# Autodesk Inventor assembly: P1704_E001
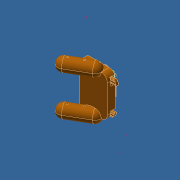
[picture p0: Inventor's stored thumbnail of the model, 180x180]
Saved by Autodesk Inventor 2019 (Build 230136000, 136)
## iProperties
Created: 2019-04-29
Part Number: P1704_E001
Material: Générique
Document SubType Name: Assembly
Designer: Joan.MAILLARD
Author: Joan.MAILLARD
## Documents named in this file (16)
- P:\projet_manette\manette\06_Dessins\2019\Manette universelle\P1704_E001.iam
- P:\projet_manette\manette\06_Dessins\2019\Manette universelle\P1704_004_mainDroiteExterieur.ipt
- P:\projet_manette\manette\06_Dessins\2019\Manette universelle\P1704_005_mainGaucheExterieur.ipt
- P:\projet_manette\manette\06_Dessins\2019\Manette universelle\P1704_001_basManette.ipt
- P:\projet_manette\manette\06_Dessins\2019\Manette universelle\P1704_006_gachette.ipt
- P:\projet_manette\manette\06_Dessins\2019\Manette universelle\P1704_007_guideRessort.ipt
- P:\projet_manette\manette\06_Dessins\2019\Manette universelle\P1704_002_mainDroiteInterieur.ipt
- P:\projet_manette\manette\06_Dessins\2019\Manette universelle\P1704_003_mainGaucheInterieur.ipt
- P:\projet_manette\manette\06_Dessins\2019\Manette universelle\P1704_009_slider.ipt
- P:\projet_manette\manette\06_Dessins\2019\Manette universelle\P1704_011_4buttonPCB.ipt
- P:\projet_manette\manette\06_Dessins\2019\Manette universelle\P1704_010_startSelectPCB.ipt
- P:\projet_manette\manette\06_Dessins\2019\Manette universelle\P1704_012_joystick.ipt
- P:\projet_manette\manette\06_Dessins\2019\Manette universelle\P1704_014_Display.ipt
- P:\projet_manette\manette\06_Dessins\2019\Manette universelle\P1704_015_rumble.ipt
- P:\projet_manette\manette\06_Dessins\2019\Manette universelle\P1704_016_Button.ipt
- P:\projet_manette\manette\06_Dessins\2019\Manette universelle\P1704_017_button_cap.ipt
## Components (21 placed, 15 different names)
1. P1704_004_mainDroiteExterieur:1 — Rotation:7, Rotation:8, Placage:14
2. P1704_005_mainGaucheExterieur:1 — Rotation:9, Rotation:10, Placage:12
3. P1704_001_basManette:1 — Placage:11, Placage:12, Placage:13, Placage:14, Placage:20, Placage:22, Placage:24, Placage:26, Placage:27, Placage:30, Placage:31, Placage:32, Placage:33, Placage:34, Placage:35, Placage:38
4. P1704_006_gachette:1 — Rotation:2, Glissière:4, Placage:26, Placage:27, Affleurement:1
5. P1704_006_gachette:2 — Rotation:1, Glissière:3
6. P1704_007_guideRessort:1 — Rotation:1
7. P1704_007_guideRessort:2 — Rotation:2
8. P1704_002_mainDroiteInterieur:1 — Rotation:7, Rotation:8, Placage:13
9. P1704_003_mainGaucheInterieur:1 — Rotation:9, Rotation:10, Placage:11
10. P1704_009_slider:1 — Glissière:3
11. P1704_009_slider:2 — Glissière:4, Affleurement:1
12. manette_2019_boutons.kicad_pcb_Contour:1 — Placage:22, Placage:36, Placage:37, Affleurement:2, Affleurement:3
13. manette_2019_boutons.kicad_pcb_Contour:2 — Placage:20
14. Manette_2019_PCB_Central.kicad_pcb_Contour:1 — Placage:24
15. P1704_012_joystick:1 — Placage:30, Placage:31
16. P1704_012_joystick:2 — Placage:32, Placage:33
17. P1704_014_Display:1 — Placage:37, Placage:38
18. P1704_015_rumble:1 — Placage:34
19. P1704_015_rumble:2 — Placage:35
20. P1704_016_Button:7 — Placage:36, Affleurement:2, Affleurement:3, Placage:39, Placage:40
21. P1704_017_button_cap:1 — Placage:39, Placage:40
## Relationships (31: Mate 20, RevoluteJoint 6, Flush 3, TranslationJoint 2)
- Rotation:1 [RevoluteJoint] (4.5 mm): P1704_006_gachette:2 ↔ P1704_007_guideRessort:1
- Rotation:2 [RevoluteJoint] (4.5 mm): P1704_006_gachette:1 ↔ P1704_007_guideRessort:2
- Rotation:7 [RevoluteJoint]: P1704_004_mainDroiteExterieur:1 ↔ P1704_002_mainDroiteInterieur:1
- Rotation:8 [RevoluteJoint]: P1704_004_mainDroiteExterieur:1 ↔ P1704_002_mainDroiteInterieur:1
- Rotation:9 [RevoluteJoint]: P1704_005_mainGaucheExterieur:1 ↔ P1704_003_mainGaucheInterieur:1
- Rotation:10 [RevoluteJoint]: P1704_005_mainGaucheExterieur:1 ↔ P1704_003_mainGaucheInterieur:1
- Glissière:3 [TranslationJoint]: P1704_006_gachette:2 ↔ P1704_009_slider:1
- Glissière:4 [TranslationJoint]: P1704_006_gachette:1 ↔ P1704_009_slider:2
- Placage:11 [Mate]: P1704_001_basManette:1 ↔ P1704_003_mainGaucheInterieur:1
- Placage:12 [Mate]: P1704_005_mainGaucheExterieur:1 ↔ P1704_001_basManette:1
- Placage:13 [Mate]: P1704_001_basManette:1 ↔ P1704_002_mainDroiteInterieur:1
- Placage:14 [Mate]: P1704_004_mainDroiteExterieur:1 ↔ P1704_001_basManette:1
- Placage:20 [Mate] (10 mm): P1704_001_basManette:1 ↔ manette_2019_boutons.kicad_pcb_Contour:2
- Placage:22 [Mate] (5 mm): P1704_001_basManette:1 ↔ manette_2019_boutons.kicad_pcb_Contour:1
- Placage:24 [Mate] (57.5375 mm): P1704_001_basManette:1 ↔ Manette_2019_PCB_Central.kicad_pcb_Contour:1
- Placage:26 [Mate]: P1704_001_basManette:1 ↔ P1704_006_gachette:1
- Placage:27 [Mate]: P1704_001_basManette:1 ↔ P1704_006_gachette:1
- Affleurement:1 [Flush]: P1704_006_gachette:1 ↔ P1704_009_slider:2
- Placage:30 [Mate] (35 mm): P1704_001_basManette:1 ↔ P1704_012_joystick:1
- Placage:31 [Mate] (40 mm): P1704_001_basManette:1 ↔ P1704_012_joystick:1
- Placage:32 [Mate] (35 mm): P1704_001_basManette:1 ↔ P1704_012_joystick:2
- Placage:33 [Mate] (35 mm): P1704_001_basManette:1 ↔ P1704_012_joystick:2
- Placage:34 [Mate]: P1704_001_basManette:1 ↔ P1704_015_rumble:1
- Placage:35 [Mate]: P1704_001_basManette:1 ↔ P1704_015_rumble:2
- Placage:36 [Mate]: manette_2019_boutons.kicad_pcb_Contour:1 ↔ P1704_016_Button:7
- Placage:37 [Mate] (6.4 mm): manette_2019_boutons.kicad_pcb_Contour:1 ↔ P1704_014_Display:1
- Placage:38 [Mate] (53.375 mm): P1704_001_basManette:1 ↔ P1704_014_Display:1
- Affleurement:2 [Flush] (5.15 mm): manette_2019_boutons.kicad_pcb_Contour:1 ↔ P1704_016_Button:7
- Affleurement:3 [Flush] (16.6 mm): manette_2019_boutons.kicad_pcb_Contour:1 ↔ P1704_016_Button:7
- Placage:39 [Mate]: P1704_016_Button:7 ↔ P1704_017_button_cap:1
- Placage:40 [Mate]: P1704_016_Button:7 ↔ P1704_017_button_cap:1
